# Autodesk Inventor assembly: Тумба ТВ
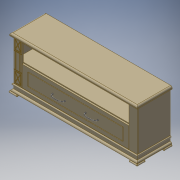
[picture p0: Inventor's stored thumbnail of the model, 180x180]
Saved by Autodesk Inventor 2019 (Build 230136000, 136)
## iProperties
Created: 2018-09-22
Part Number: Тумба ТВ
Material: Типовые
Document SubType Name: Assembly
Designer: Андреев Н.Л.
Mass: 57745.9 g
Surface Area: 81947.1 cm^2
Volume: 79749.9 cm^3
Density: 0.724088 g/cm^3
Author: Андреев Н.Л.
## Documents named in this file (14)
- C:\Users\andrnl\Documents\Inventor\Мурзин\Тумба ТВ.iam
- C:\Users\andrnl\Documents\Inventor\Мурзин\ТВ Стенка боковая.ipt
- C:\Users\andrnl\Documents\Inventor\Мурзин\Твердое тело10.ipt
- C:\Users\andrnl\Documents\Inventor\Мурзин\ТВ Стенка задняя.ipt
- C:\Users\andrnl\Documents\Inventor\Мурзин\ТВ Пилястра.ipt
- C:\Users\andrnl\Documents\Inventor\Мурзин\Твердое тело15.ipt
- C:\Users\andrnl\Documents\Inventor\Мурзин\ТВ Фасад ящика.ipt
- C:\Users\andrnl\Documents\Inventor\Мурзин\ТВ Дно.ipt
- C:\Users\andrnl\Documents\Inventor\Мурзин\ТВ Цоколь.ipt
- C:\Users\andrnl\Documents\Inventor\Мурзин\ТВ Ножка.ipt
- C:\Users\andrnl\Documents\Inventor\Мурзин\ТВ Планка цоколя.ipt
- C:\Users\andrnl\Documents\Inventor\Мурзин\ТВ Полка.ipt
- C:\Users\andrnl\Documents\Inventor\Мурзин\ТВ Столешница.ipt
- C:\Users\andrnl\Documents\Inventor\Мурзин\Ручка скоба.ipt
## Components (17 placed, 13 different names)
1. ТВ Стенка боковая:1
2. Твердое тело10:1
3. ТВ Стенка задняя:1
4. ТВ Пилястра:1
5. Твердое тело15:1
6. ТВ Фасад ящика:1 — Совмещение:1, Совмещение:2
7. ТВ Дно:1
8. ТВ Цоколь:1
9. ТВ Планка цоколя:1
10. ТВ Полка:1
11. ТВ Столешница:1
12. Ручка скоба:1 — Совмещение:1, Совмещение:2, Совмещение:3
13. Ручка скоба:2 — Заподлицо:1
14. ТВ Ножка:1
15. ТВ Ножка:2
16. ТВ Ножка:3
17. ТВ Ножка:4
## Component patterns: (2 elements, first: ТВ Ножка:1 + ТВ Ножка:2)
## Relationships (4: Mate 3, Flush 1)
- Совмещение:1 [Mate]: ТВ Фасад ящика:1 ↔ Ручка скоба:1
- Совмещение:2 [Mate]: ТВ Фасад ящика:1 ↔ Ручка скоба:1
- Совмещение:3 [Mate] (200 mm): Ручка скоба:1
- Заподлицо:1 [Flush] (200 mm): Ручка скоба:2
